# Autodesk Inventor assembly: SensorLamp
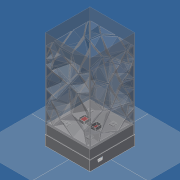
[picture p0: Inventor's stored thumbnail of the model, 180x180]
Saved by Autodesk Inventor 2016 SP2 (Build 200236200, 236)
## iProperties
Created: 2017-11-09
Part Number: SensorLamp
Material: Generisch
Document SubType Name: Assembly
Designer: User
Author: User
## Documents named in this file (8)
- C:\Users\User\Documents\Inventor\SensorLamp\SensorLamp.iam
- C:\Users\User\Documents\Inventor\SensorLamp\SharpDistanceRanger.ipt
- C:\Users\User\Documents\Inventor\SensorLamp\arduino-nano-v3\NanoV3 v4.iam
- C:\Users\User\Documents\Inventor\SensorLamp\led-super-flux\7676C.ipt
- C:\Users\User\Documents\Inventor\SensorLamp\Sensorlamp_Base.ipt
- C:\Users\User\Documents\Inventor\SensorLamp\Sensorlamp_Cover.ipt
- C:\Users\User\Documents\Inventor\SensorLamp\PCB_70x30.ipt
- C:\Users\User\Documents\Inventor\SensorLamp\lamp-shade\crinklelamp_hollow_topless_scaled.ipt
## Components (10 placed, 7 different names)
1. SharpDistanceRanger:1 — Passend:11, Passend:12, Passend:13
2. NanoV3 v4:1 [sub-assembly] — Passend:1, Passend:24, Winkel:1
3. Sensorlamp_Base:1 — Fluchtend:19, Fluchtend:20, Passend:21, Passend:22, Passend:23, Passend:25, Fluchtend:21, Fluchtend:22, Passend:26
4. Sensorlamp_Cover:1 — Passend:11, Passend:12, Passend:13, Passend:14, Passend:15, Passend:16, Passend:17, Fluchtend:19, Fluchtend:20, Passend:25
5. PCB_70x30:2 — Passend:1, Passend:21, Passend:22, Passend:23, Passend:24, Winkel:1
6. 7676C:1 — Passend:16
7. 7676C:2 — Passend:14
8. 7676C:3 — Passend:15
9. 7676C:4 — Passend:17
10. crinklelamp_hollow_topless_scaled:1 — Fluchtend:21, Fluchtend:22, Passend:26
## Relationships (19: Mate 14, Flush 4, Angle 1)
- Passend:1 [Mate] (-10 mm): NanoV3 v4:1 ↔ PCB_70x30:2
- Passend:11 [Mate]: SharpDistanceRanger:1 ↔ Sensorlamp_Cover:1
- Passend:12 [Mate]: SharpDistanceRanger:1 ↔ Sensorlamp_Cover:1
- Passend:13 [Mate]: SharpDistanceRanger:1 ↔ Sensorlamp_Cover:1
- Passend:14 [Mate]: Sensorlamp_Cover:1 ↔ 7676C:2
- Passend:15 [Mate]: Sensorlamp_Cover:1 ↔ 7676C:3
- Passend:16 [Mate]: Sensorlamp_Cover:1 ↔ 7676C:1
- Passend:17 [Mate]: Sensorlamp_Cover:1 ↔ 7676C:4
- Fluchtend:19 [Flush]: Sensorlamp_Base:1 ↔ Sensorlamp_Cover:1
- Fluchtend:20 [Flush]: Sensorlamp_Base:1 ↔ Sensorlamp_Cover:1
- Passend:21 [Mate]: Sensorlamp_Base:1 ↔ PCB_70x30:2
- Passend:22 [Mate]: Sensorlamp_Base:1 ↔ PCB_70x30:2
- Passend:23 [Mate]: Sensorlamp_Base:1 ↔ PCB_70x30:2
- Passend:24 [Mate]: NanoV3 v4:1 ↔ PCB_70x30:2
- Winkel:1 [Angle] (0 deg): NanoV3 v4:1 ↔ PCB_70x30:2
- Passend:25 [Mate]: Sensorlamp_Base:1 ↔ Sensorlamp_Cover:1
- Fluchtend:21 [Flush]: Sensorlamp_Base:1 ↔ crinklelamp_hollow_topless_scaled:1
- Fluchtend:22 [Flush]: Sensorlamp_Base:1 ↔ crinklelamp_hollow_topless_scaled:1
- Passend:26 [Mate]: Sensorlamp_Base:1 ↔ crinklelamp_hollow_topless_scaled:1
